# Autodesk Inventor assembly: Assembly
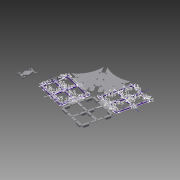
[picture p0: Inventor's stored thumbnail of the model, 180x180]
Saved by Autodesk Inventor 2014 SP1 (Build 180222100, 222)
## iProperties
Created: 2015-03-29
Part Number: Assembly
Document SubType Name: Assembly
Designer: Erin
Author: Erin
## Documents named in this file (9)
- C:\Users\Erin\Desktop\RDAS Base\Assembly.iam
- C:\Users\Erin\Desktop\RDAS Base\Base.ipt
- C:\Users\Erin\Desktop\RDAS Base\SideLink.ipt
- C:\Users\Erin\Desktop\RDAS Base\Side.ipt
- C:\Users\Erin\Desktop\RDAS Base\SolarLink.ipt
- C:\Users\Erin\Desktop\RDAS Base\SolarPanel_A.ipt
- C:\Users\Erin\Desktop\RDAS Base\SolarPanel_B.ipt
- C:\Users\Erin\Desktop\RDAS Base\SnapConnector.ipt
- C:\Users\Erin\Desktop\RDAS Base\SnapInsert.ipt
## Components (12 placed, 8 different names)
1. Base:1 — Insert:1, Insert:4, Insert:5, Insert:19
2. SideLink:1 — Insert:1, Insert:2, Insert:3, Insert:19
3. SideLink:2 — Insert:4, Insert:5, Insert:6, Insert:7
4. Side:1 — Insert:2, Insert:3, Insert:8, Insert:9, Insert:22, Insert:23, Flush:1
5. Side:2 — Insert:6, Insert:7, Insert:10, Insert:11
6. SolarLink:1 — Insert:8, Insert:9, Insert:12, Insert:13
7. SolarPanel_A:1 — Insert:12, Insert:13, Insert:14, Insert:15, Insert:16
8. SolarPanel_B:1 — Insert:17, Insert:18, Insert:20, Insert:21
9. SolarLink:2 — Insert:10, Insert:11, Insert:17, Insert:18
10. SolarLink:3 — Insert:14, Insert:15, Insert:16, Insert:20, Insert:21
11. SnapConnector:1
12. SnapInsert:1 — Insert:22, Insert:23, Flush:1
## Relationships (24: Insert 23, Flush 1)
- Insert:1: Base:1 ↔ SideLink:1
- Insert:2: SideLink:1 ↔ Side:1
- Insert:3: SideLink:1 ↔ Side:1
- Insert:4: Base:1 ↔ SideLink:2
- Insert:5: Base:1 ↔ SideLink:2
- Insert:6: SideLink:2 ↔ Side:2
- Insert:7: SideLink:2 ↔ Side:2
- Insert:8: Side:1 ↔ SolarLink:1
- Insert:9: Side:1 ↔ SolarLink:1
- Insert:10: Side:2 ↔ SolarLink:2
- Insert:11: Side:2 ↔ SolarLink:2
- Insert:12: SolarLink:1 ↔ SolarPanel_A:1
- Insert:13: SolarLink:1 ↔ SolarPanel_A:1
- Insert:14: SolarPanel_A:1 ↔ SolarLink:3
- Insert:15: SolarPanel_A:1 ↔ SolarLink:3
- Insert:16: SolarPanel_A:1 ↔ SolarLink:3
- Insert:17: SolarPanel_B:1 ↔ SolarLink:2
- Insert:18: SolarPanel_B:1 ↔ SolarLink:2
- Insert:19: Base:1 ↔ SideLink:1
- Insert:20: SolarPanel_B:1 ↔ SolarLink:3
- Insert:21: SolarPanel_B:1 ↔ SolarLink:3
- Insert:22: Side:1 ↔ SnapInsert:1
- Insert:23: Side:1 ↔ SnapInsert:1
- Flush:1: Side:1 ↔ SnapInsert:1
